# Autodesk Inventor assembly: ZB_Temperierstation
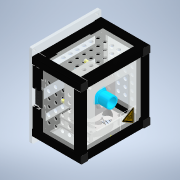
[picture p0: Inventor's stored thumbnail of the model, 180x180]
Saved by Autodesk Inventor 2022 (Build 260153000, 153)
## iProperties
Created: 2021-05-07
Part Number: ZB_Temperierstation
Document SubType Name: Assembly
Designer: Sebastian Seewald
Sending System: Autodesk Inventor 2021
Preprocessor: ST-DEVELOPER v18.1
Title: C:\Users\Sebastian Seewald\Documents\Inventor\Konstruktion_Studium\Projekt_1\Temperiereinheit\ZB\ZB_Temperierstation.stp
Author: Sebastian Seewald
## Documents named in this file (28)
- E:\Transfer\Sync\Hivemind\1-MCI-Unterlagen\Master\Semester 3\Projekt 2\011_Kartesischer_Roboter_Modul\07-CAD Files\03-Heizelement\ZB_Temperierstation.iam
- E:\Transfer\Sync\Hivemind\1-MCI-Unterlagen\Master\Semester 3\Projekt 2\011_Kartesischer_Roboter_Modul\07-CAD Files\03-Heizelement\0001_flasche.ipt
- E:\Transfer\Sync\Hivemind\1-MCI-Unterlagen\Master\Semester 3\Projekt 2\011_Kartesischer_Roboter_Modul\07-CAD Files\03-Heizelement\Temperierblock.ipt
- E:\Transfer\Sync\Hivemind\1-MCI-Unterlagen\Master\Semester 3\Projekt 2\011_Kartesischer_Roboter_Modul\07-CAD Files\03-Heizelement\Keramikhülse.ipt
- E:\Transfer\Sync\Hivemind\1-MCI-Unterlagen\Master\Semester 3\Projekt 2\011_Kartesischer_Roboter_Modul\07-CAD Files\03-Heizelement\ITEM_20x20_N2_200mm.ipt
- E:\Transfer\Sync\Hivemind\1-MCI-Unterlagen\Master\Semester 3\Projekt 2\011_Kartesischer_Roboter_Modul\07-CAD Files\03-Heizelement\Schutzglas.ipt
- E:\Transfer\Sync\Hivemind\1-MCI-Unterlagen\Master\Semester 3\Projekt 2\011_Kartesischer_Roboter_Modul\07-CAD Files\03-Heizelement\Schutzglas_oben.ipt
- E:\Transfer\Sync\Hivemind\1-MCI-Unterlagen\Master\Semester 3\Projekt 2\011_Kartesischer_Roboter_Modul\07-CAD Files\03-Heizelement\Schutzglas_Lüfter.ipt
- E:\Transfer\Sync\Hivemind\1-MCI-Unterlagen\Master\Semester 3\Projekt 2\011_Kartesischer_Roboter_Modul\07-CAD Files\03-Heizelement\3412ngh-rs0.ipt
- E:\Transfer\Sync\Hivemind\1-MCI-Unterlagen\Master\Semester 3\Projekt 2\011_Kartesischer_Roboter_Modul\07-CAD Files\03-Heizelement\Bimetallschalter.ipt
- E:\Transfer\Sync\Hivemind\1-MCI-Unterlagen\Master\Semester 3\Projekt 2\011_Kartesischer_Roboter_Modul\07-CAD Files\03-Heizelement\Distanzhülse.ipt
- E:\Transfer\Sync\Hivemind\1-MCI-Unterlagen\Master\Semester 3\Projekt 2\011_Kartesischer_Roboter_Modul\07-CAD Files\03-Heizelement\din_912-m4x0_7-35-10_9.ipt
- E:\Transfer\Sync\Hivemind\1-MCI-Unterlagen\Master\Semester 3\Projekt 2\011_Kartesischer_Roboter_Modul\07-CAD Files\03-Heizelement\mutter_din_934-m4x0_7.ipt
- E:\Transfer\Sync\Hivemind\1-MCI-Unterlagen\Master\Semester 3\Projekt 2\011_Kartesischer_Roboter_Modul\07-CAD Files\03-Heizelement\Schutzgitter.ipt
- E:\Transfer\Sync\Hivemind\1-MCI-Unterlagen\Master\Semester 3\Projekt 2\011_Kartesischer_Roboter_Modul\07-CAD Files\03-Heizelement\din_912-m3x0_5-6-10_9.ipt
- E:\Transfer\Sync\Hivemind\1-MCI-Unterlagen\Master\Semester 3\Projekt 2\011_Kartesischer_Roboter_Modul\07-CAD Files\03-Heizelement\HP_8x60_160W.ipt
- E:\Transfer\Sync\Hivemind\1-MCI-Unterlagen\Master\Semester 3\Projekt 2\011_Kartesischer_Roboter_Modul\07-CAD Files\03-Heizelement\Thermoelement.ipt
- E:\Transfer\Sync\Hivemind\1-MCI-Unterlagen\Master\Semester 3\Projekt 2\011_Kartesischer_Roboter_Modul\07-CAD Files\03-Heizelement\Abdeckkappe 5 20x20.ipt
- E:\Transfer\Sync\Hivemind\1-MCI-Unterlagen\Master\Semester 3\Projekt 2\011_Kartesischer_Roboter_Modul\07-CAD Files\03-Heizelement\Unterlegscheiben_Keramik.ipt
- E:\Transfer\Sync\Hivemind\1-MCI-Unterlagen\Master\Semester 3\Projekt 2\011_Kartesischer_Roboter_Modul\07-CAD Files\03-Heizelement\din_913-m4x10-c3.ipt
- E:\Transfer\Sync\Hivemind\1-MCI-Unterlagen\Master\Semester 3\Projekt 2\011_Kartesischer_Roboter_Modul\07-CAD Files\03-Heizelement\din_913-m4x8-a4.ipt
- E:\Transfer\Sync\Hivemind\1-MCI-Unterlagen\Master\Semester 3\Projekt 2\011_Kartesischer_Roboter_Modul\07-CAD Files\03-Heizelement\ITEM_20x20_N2_180mm.ipt
- E:\Transfer\Sync\Hivemind\1-MCI-Unterlagen\Master\Semester 3\Projekt 2\011_Kartesischer_Roboter_Modul\07-CAD Files\03-Heizelement\ITEM_20x20_N1_200mm.ipt
- E:\Transfer\Sync\Hivemind\1-MCI-Unterlagen\Master\Semester 3\Projekt 2\011_Kartesischer_Roboter_Modul\07-CAD Files\03-Heizelement\ITEM_20x20_200mm_Montage.ipt
- E:\Transfer\Sync\Hivemind\1-MCI-Unterlagen\Master\Semester 3\Projekt 2\011_Kartesischer_Roboter_Modul\07-CAD Files\03-Heizelement\Beilagscheibe_M5x1.ipt
- E:\Transfer\Sync\Hivemind\1-MCI-Unterlagen\Master\Semester 3\Projekt 2\011_Kartesischer_Roboter_Modul\07-CAD Files\03-Heizelement\ITEM_20x20_77mm.ipt
- E:\Transfer\Sync\Hivemind\1-MCI-Unterlagen\Master\Semester 3\Projekt 2\011_Kartesischer_Roboter_Modul\07-CAD Files\03-Heizelement\Kabeldurchführung.ipt
- E:\Transfer\Sync\Hivemind\1-MCI-Unterlagen\Master\Semester 3\Projekt 2\011_Kartesischer_Roboter_Modul\07-CAD Files\03-Heizelement\Heizelement_Grundplatte.ipt
## Components (73 placed, 27 different names)
1. Temperierblock:1 — Passend:48, Passend:176, Passend:177, Passend:178, Passend:179, Passend:180, Passend:181, Fluchtend:52, Fluchtend:53, Fluchtend:54, Fluchtend:55, Fluchtend:56, Fluchtend:57, Passend:182, Passend:184, Passend:187, Passend:188, Passend:189, Passend:231, Passend:251, Passend:258, Passend:259, Passend:260, Passend:261, Passend:262, Passend:263, Passend:264, Passend:303, Passend:304, Passend:305, Passend:306, Passend:307
2. Keramikhülse:1 — Passend:48, Passend:258, Passend:269, Passend:284
3. Keramikhülse:2 — Passend:263, Passend:264, Passend:265
4. Keramikhülse:3 — Passend:259, Passend:260, Passend:296
5. Keramikhülse:4 — Passend:261, Passend:262, Passend:266, Passend:288
6. Schutzglas:1 — Passend:212, Mate:249, Passend:250, Passend:308, Passend:309
7. Schutzglas:2 — Passend:215, Passend:245, Passend:246
8. Schutzglas:3 — Passend:214, Passend:247, Passend:248
9. ITEM_20x20_N2_200mm:8 — Passend:61, Passend:195, Passend:196, Fluchtend:63, Passend:240, Passend:241, Fluchtend:97, Passend:248
10. ITEM_20x20_N2_200mm:9 — Passend:62, Passend:193, Fluchtend:58, Fluchtend:60, Passend:242, Passend:243
11. ITEM_20x20_N2_200mm:10 — Passend:60, Passend:205, Fluchtend:76, Fluchtend:77, Passend:244
12. ITEM_20x20_N2_200mm:11 — Fluchtend:24, Passend:206, Fluchtend:78, Fluchtend:79, Passend:237, Passend:238, Passend:250
13. Schutzglas_oben:1 — Passend:60, Passend:61, Passend:62
14. Schutzglas_Lüfter:1 — Passend:118, Passend:119, Passend:120, Passend:121, Passend:122, Passend:123, Passend:124, Passend:129, Passend:130, Passend:131, Passend:132, Tangential:1, Passend:210, Passend:280, Passend:281
15. 3412ngh-rs0:1 — Passend:118, Passend:119, Passend:120, Passend:125, Passend:126, Passend:127, Passend:128, Passend:139, Passend:140, Passend:141, Passend:163
16. Bimetallschalter:1 — Passend:104, Passend:105, Passend:106, Passend:107, Passend:305
17. Distanzhülse:1 — Passend:121, Passend:126
18. Distanzhülse:2 — Passend:122, Passend:125
19. Distanzhülse:3 — Passend:123, Passend:128
20. Distanzhülse:4 — Passend:124, Passend:127
21. din_912-m4x0_7-35-10_9:1 — Passend:129, Tangential:2, Passend:135
22. din_912-m4x0_7-35-10_9:2 — Passend:132, Passend:134, Tangential:4, Passend:138
23. din_912-m4x0_7-35-10_9:3 — Passend:130, Passend:133, Tangential:3, Passend:136
24. din_912-m4x0_7-35-10_9:4 — Passend:131, Tangential:5, Passend:137
25. din_934-m4x0_7:1 — Passend:138, Passend:139
26. din_934-m4x0_7:2 — Passend:135, Passend:140
27. din_934-m4x0_7:3 — Passend:136, Passend:141
28. din_934-m4x0_7:4 — Passend:137, Passend:163
29. Schutzgitter:1 — Passend:133, Passend:134, Tangential:1, Tangential:2, Tangential:3, Tangential:4, Tangential:5
30. din_912-m3x0_5-6-10_9:1 — Passend:104, Passend:107, Passend:306
31. din_912-m3x0_5-6-10_9:2 — Passend:105, Passend:106, Passend:307
32. HP_8x60_160W:1 — Passend:176, Fluchtend:54, Tangential:6
33. HP_8x60_160W:2 — Passend:178, Fluchtend:57, Tangential:9
34. HP_8x60_160W:3 — Passend:177, Fluchtend:52, Tangential:7
35. HP_8x60_160W:4 — Passend:179, Fluchtend:55, Tangential:12
36. Thermoelement:1 — Passend:181, Fluchtend:53, Tangential:11
37. Thermoelement:2 — Passend:180, Fluchtend:56, Tangential:10
38. Abdeckkappe 5 20x20:1 — Passend:194, Fluchtend:61, Fluchtend:62
39. Abdeckkappe 5 20x20:2 — Fluchtend:24, Passend:207, Fluchtend:83, Fluchtend:84
40. Abdeckkappe 5 20x20:3 — Passend:209, Fluchtend:87, Fluchtend:88
41. Abdeckkappe 5 20x20:4 — Passend:208, Fluchtend:85, Fluchtend:86
42. Unterlegscheiben_Keramik:1 — Passend:275, Passend:294, Passend:297, Passend:302
43. Unterlegscheiben_Keramik:2 — Passend:274, Passend:295, Passend:299, Passend:300
44. Unterlegscheiben_Keramik:3 — Passend:273, Passend:289, Passend:290, Passend:298, Passend:301
45. Unterlegscheiben_Keramik:4 — Passend:272, Passend:291, Passend:292, Passend:293
46. din_913-m4x10-c3:2 — Passend:187, Tangential:9
47. din_913-m4x10-c3:4 — Passend:184, Tangential:7
48. din_913-m4x10-c3:5 — Passend:182, Tangential:6
49. din_913-m4x10-c3:6 — Passend:231, Tangential:12
50. din_913-m4x8-a4:1 — Passend:189, Tangential:11
51. din_913-m4x8-a4:2 — Passend:188, Tangential:10
52. ITEM_20x20_N2_180mm:1 — Passend:209, Fluchtend:87, Fluchtend:88, Passend:242, Passend:243, Passend:244, Passend:245, Passend:279, Fluchtend:101, Fluchtend:102, Mate:312
53. ITEM_20x20_N2_180mm:2 — Passend:193, Fluchtend:58, Fluchtend:60, Passend:194, Fluchtend:61, Fluchtend:62, Passend:195, Passend:196, Fluchtend:63, Passend:215, Passend:232, Fluchtend:89, Fluchtend:90, Passend:233, Fluchtend:91, Fluchtend:92, Mate:313
54. ITEM_20x20_N2_180mm:3 — Passend:207, Fluchtend:83, Fluchtend:84, Passend:214, Passend:237, Passend:238, Passend:240, Passend:241, Fluchtend:97, Passend:283, Fluchtend:105, Fluchtend:106
55. ITEM_20x20_N2_180mm:4 — Passend:205, Fluchtend:76, Fluchtend:77, Passend:206, Fluchtend:78, Fluchtend:79, Passend:208, Fluchtend:85, Fluchtend:86, Passend:210, Passend:212, Mate:249, Passend:280, Passend:282, Fluchtend:103, Fluchtend:104
56. ITEM_20x20_N1_200mm:1 — Passend:232, Fluchtend:89, Fluchtend:90, Passend:246, Passend:285, Passend:286, Fluchtend:107, Fluchtend:108, Mate:311
57. ITEM_20x20_N1_200mm:2 — Passend:279, Fluchtend:101, Fluchtend:102, Passend:281
58. ITEM_20x20_N1_200mm:3 — Passend:233, Fluchtend:91, Fluchtend:92, Passend:247, Passend:251, Mate:253
59. ITEM_20x20_200mm_Montage:1 — Mate:253, Passend:256, Passend:268, Passend:272, Passend:275, Passend:285, Fluchtend:108, Passend:291, Passend:292, Passend:294
60. ITEM_20x20_200mm_Montage:2 — Passend:257, Passend:267, Passend:273, Passend:274, Passend:286, Fluchtend:107, Passend:288, Passend:289, Passend:290, Passend:295
61. Beilagscheibe_M5x1:1 — Passend:256, Passend:269
62. Beilagscheibe_M5x1:2 — Passend:257, Passend:296
63. Beilagscheibe_M5x1:3 — Passend:265, Passend:268
64. Beilagscheibe_M5x1:4 — Passend:266, Passend:267
65. ITEM_20x20_77mm:1 — Passend:283, Fluchtend:105, Fluchtend:106
66. ITEM_20x20_77mm:2 — Passend:282, Fluchtend:103, Fluchtend:104, Passend:310
67. din_912-m4x0_7-35-10_9:5 — Passend:284, Passend:293
68. din_912-m4x0_7-35-10_9:6 — Passend:298, Passend:301
69. din_912-m4x0_7-35-10_9:7 — Passend:299, Passend:300
70. din_912-m4x0_7-35-10_9:8 — Passend:297, Passend:302
71. 0001_flasche:1 — Passend:303, Passend:304
72. Kabeldurchführung:1 — Passend:308, Passend:309, Passend:310
73. Heizelement_Grundplatte:1 — Mate:311, Mate:312, Mate:313
## Relationships (173: Mate 127, Flush 35, Tangent 11)
- Passend:48 [Mate]: Temperierblock:1 ↔ Keramikhülse:1
- Fluchtend:24 [Flush]: ITEM_20x20_N2_200mm:11 ↔ Abdeckkappe 5 20x20:2
- Passend:60 [Mate]: ITEM_20x20_N2_200mm:10 ↔ Schutzglas_oben:1
- Passend:61 [Mate]: ITEM_20x20_N2_200mm:8 ↔ Schutzglas_oben:1
- Passend:62 [Mate]: ITEM_20x20_N2_200mm:9 ↔ Schutzglas_oben:1
- Passend:104 [Mate]: Bimetallschalter:1 ↔ din_912-m3x0_5-6-10_9:1
- Passend:105 [Mate]: Bimetallschalter:1 ↔ din_912-m3x0_5-6-10_9:2
- Passend:106 [Mate]: Bimetallschalter:1 ↔ din_912-m3x0_5-6-10_9:2
- Passend:107 [Mate]: Bimetallschalter:1 ↔ din_912-m3x0_5-6-10_9:1
- Passend:118 [Mate]: Schutzglas_Lüfter:1 ↔ 3412ngh-rs0:1
- Passend:119 [Mate]: Schutzglas_Lüfter:1 ↔ 3412ngh-rs0:1
- Passend:120 [Mate]: Schutzglas_Lüfter:1 ↔ 3412ngh-rs0:1
- Passend:121 [Mate]: Schutzglas_Lüfter:1 ↔ Distanzhülse:1
- Passend:122 [Mate]: Schutzglas_Lüfter:1 ↔ Distanzhülse:2
- Passend:123 [Mate]: Schutzglas_Lüfter:1 ↔ Distanzhülse:3
- Passend:124 [Mate]: Schutzglas_Lüfter:1 ↔ Distanzhülse:4
- Passend:125 [Mate]: 3412ngh-rs0:1 ↔ Distanzhülse:2
- Passend:126 [Mate]: 3412ngh-rs0:1 ↔ Distanzhülse:1
- Passend:127 [Mate]: 3412ngh-rs0:1 ↔ Distanzhülse:4
- Passend:128 [Mate]: 3412ngh-rs0:1 ↔ Distanzhülse:3
- Passend:129 [Mate]: Schutzglas_Lüfter:1 ↔ din_912-m4x0_7-35-10_9:1
- Passend:130 [Mate]: Schutzglas_Lüfter:1 ↔ din_912-m4x0_7-35-10_9:3
- Passend:131 [Mate]: Schutzglas_Lüfter:1 ↔ din_912-m4x0_7-35-10_9:4
- Passend:132 [Mate]: Schutzglas_Lüfter:1 ↔ din_912-m4x0_7-35-10_9:2
- Passend:133 [Mate]: din_912-m4x0_7-35-10_9:3 ↔ Schutzgitter:1
- Passend:134 [Mate]: din_912-m4x0_7-35-10_9:2 ↔ Schutzgitter:1
- Tangential:1: Schutzglas_Lüfter:1 ↔ Schutzgitter:1
- Tangential:2: din_912-m4x0_7-35-10_9:1 ↔ Schutzgitter:1
- Tangential:3: din_912-m4x0_7-35-10_9:3 ↔ Schutzgitter:1
- Tangential:4: din_912-m4x0_7-35-10_9:2 ↔ Schutzgitter:1
- Tangential:5: din_912-m4x0_7-35-10_9:4 ↔ Schutzgitter:1
- Passend:135 [Mate]: din_912-m4x0_7-35-10_9:1 ↔ din_934-m4x0_7:2
- Passend:136 [Mate]: din_912-m4x0_7-35-10_9:3 ↔ din_934-m4x0_7:3
- Passend:137 [Mate]: din_912-m4x0_7-35-10_9:4 ↔ din_934-m4x0_7:4
- Passend:138 [Mate]: din_912-m4x0_7-35-10_9:2 ↔ din_934-m4x0_7:1
- Passend:139 [Mate]: 3412ngh-rs0:1 ↔ din_934-m4x0_7:1
- Passend:140 [Mate]: 3412ngh-rs0:1 ↔ din_934-m4x0_7:2
- Passend:141 [Mate]: 3412ngh-rs0:1 ↔ din_934-m4x0_7:3
- Passend:163 [Mate]: 3412ngh-rs0:1 ↔ din_934-m4x0_7:4
- Passend:176 [Mate]: Temperierblock:1 ↔ HP_8x60_160W:1
- Passend:177 [Mate]: Temperierblock:1 ↔ HP_8x60_160W:3
- Passend:178 [Mate]: Temperierblock:1 ↔ HP_8x60_160W:2
- Passend:179 [Mate]: Temperierblock:1 ↔ HP_8x60_160W:4
- Passend:180 [Mate]: Temperierblock:1 ↔ Thermoelement:2
- Passend:181 [Mate]: Temperierblock:1 ↔ Thermoelement:1
- Fluchtend:52 [Flush]: Temperierblock:1 ↔ HP_8x60_160W:3
- Fluchtend:53 [Flush]: Temperierblock:1 ↔ Thermoelement:1
- Fluchtend:54 [Flush]: Temperierblock:1 ↔ HP_8x60_160W:1
- Fluchtend:55 [Flush]: Temperierblock:1 ↔ HP_8x60_160W:4
- Fluchtend:56 [Flush]: Temperierblock:1 ↔ Thermoelement:2
- Fluchtend:57 [Flush]: Temperierblock:1 ↔ HP_8x60_160W:2
- Passend:182 [Mate]: Temperierblock:1 ↔ din_913-m4x10-c3:5
- Passend:184 [Mate]: Temperierblock:1 ↔ din_913-m4x10-c3:4
- Passend:187 [Mate]: Temperierblock:1 ↔ din_913-m4x10-c3:2
- Tangential:6: HP_8x60_160W:1 ↔ din_913-m4x10-c3:5
- Tangential:7: HP_8x60_160W:3 ↔ din_913-m4x10-c3:4
- Tangential:9: HP_8x60_160W:2 ↔ din_913-m4x10-c3:2
- Passend:188 [Mate]: Temperierblock:1 ↔ din_913-m4x8-a4:2
- Passend:189 [Mate]: Temperierblock:1 ↔ din_913-m4x8-a4:1
- Tangential:10: Thermoelement:2 ↔ din_913-m4x8-a4:2
- Tangential:11: Thermoelement:1 ↔ din_913-m4x8-a4:1
- Passend:193 [Mate]: ITEM_20x20_N2_200mm:9 ↔ ITEM_20x20_N2_180mm:2
- Fluchtend:58 [Flush]: ITEM_20x20_N2_200mm:9 ↔ ITEM_20x20_N2_180mm:2
- Fluchtend:60 [Flush]: ITEM_20x20_N2_200mm:9 ↔ ITEM_20x20_N2_180mm:2
- Passend:194 [Mate]: Abdeckkappe 5 20x20:1 ↔ ITEM_20x20_N2_180mm:2
- Fluchtend:61 [Flush]: Abdeckkappe 5 20x20:1 ↔ ITEM_20x20_N2_180mm:2
- Fluchtend:62 [Flush]: Abdeckkappe 5 20x20:1 ↔ ITEM_20x20_N2_180mm:2
- Passend:195 [Mate]: ITEM_20x20_N2_200mm:8 ↔ ITEM_20x20_N2_180mm:2
- Passend:196 [Mate]: ITEM_20x20_N2_200mm:8 ↔ ITEM_20x20_N2_180mm:2
- Fluchtend:63 [Flush]: ITEM_20x20_N2_200mm:8 ↔ ITEM_20x20_N2_180mm:2
- Passend:205 [Mate]: ITEM_20x20_N2_200mm:10 ↔ ITEM_20x20_N2_180mm:4
- Fluchtend:76 [Flush]: ITEM_20x20_N2_200mm:10 ↔ ITEM_20x20_N2_180mm:4
- Fluchtend:77 [Flush]: ITEM_20x20_N2_200mm:10 ↔ ITEM_20x20_N2_180mm:4
- Passend:206 [Mate]: ITEM_20x20_N2_200mm:11 ↔ ITEM_20x20_N2_180mm:4
- Fluchtend:78 [Flush]: ITEM_20x20_N2_200mm:11 ↔ ITEM_20x20_N2_180mm:4
- Fluchtend:79 [Flush]: ITEM_20x20_N2_200mm:11 ↔ ITEM_20x20_N2_180mm:4
- Passend:207 [Mate]: Abdeckkappe 5 20x20:2 ↔ ITEM_20x20_N2_180mm:3
- Fluchtend:83 [Flush]: Abdeckkappe 5 20x20:2 ↔ ITEM_20x20_N2_180mm:3
- Fluchtend:84 [Flush]: Abdeckkappe 5 20x20:2 ↔ ITEM_20x20_N2_180mm:3
- Passend:208 [Mate]: Abdeckkappe 5 20x20:4 ↔ ITEM_20x20_N2_180mm:4
- Fluchtend:85 [Flush]: Abdeckkappe 5 20x20:4 ↔ ITEM_20x20_N2_180mm:4
- Fluchtend:86 [Flush]: Abdeckkappe 5 20x20:4 ↔ ITEM_20x20_N2_180mm:4
- Passend:209 [Mate]: Abdeckkappe 5 20x20:3 ↔ ITEM_20x20_N2_180mm:1
- Fluchtend:87 [Flush]: Abdeckkappe 5 20x20:3 ↔ ITEM_20x20_N2_180mm:1
- Fluchtend:88 [Flush]: Abdeckkappe 5 20x20:3 ↔ ITEM_20x20_N2_180mm:1
- Passend:210 [Mate]: Schutzglas_Lüfter:1 ↔ ITEM_20x20_N2_180mm:4
- Passend:212 [Mate]: Schutzglas:1 ↔ ITEM_20x20_N2_180mm:4
- Passend:214 [Mate]: Schutzglas:3 ↔ ITEM_20x20_N2_180mm:3
- Passend:215 [Mate]: Schutzglas:2 ↔ ITEM_20x20_N2_180mm:2
- Passend:231 [Mate]: Temperierblock:1 ↔ din_913-m4x10-c3:6
- Tangential:12: HP_8x60_160W:4 ↔ din_913-m4x10-c3:6
- Passend:232 [Mate]: ITEM_20x20_N2_180mm:2 ↔ ITEM_20x20_N1_200mm:1
- Fluchtend:89 [Flush]: ITEM_20x20_N2_180mm:2 ↔ ITEM_20x20_N1_200mm:1
- Fluchtend:90 [Flush]: ITEM_20x20_N2_180mm:2 ↔ ITEM_20x20_N1_200mm:1
- Passend:233 [Mate]: ITEM_20x20_N2_180mm:2 ↔ ITEM_20x20_N1_200mm:3
- Fluchtend:91 [Flush]: ITEM_20x20_N2_180mm:2 ↔ ITEM_20x20_N1_200mm:3
- Fluchtend:92 [Flush]: ITEM_20x20_N2_180mm:2 ↔ ITEM_20x20_N1_200mm:3
- Passend:237 [Mate]: ITEM_20x20_N2_200mm:11 ↔ ITEM_20x20_N2_180mm:3
- Passend:238 [Mate]: ITEM_20x20_N2_200mm:11 ↔ ITEM_20x20_N2_180mm:3
- Passend:240 [Mate]: ITEM_20x20_N2_200mm:8 ↔ ITEM_20x20_N2_180mm:3
- Passend:241 [Mate]: ITEM_20x20_N2_200mm:8 ↔ ITEM_20x20_N2_180mm:3
- Fluchtend:97 [Flush]: ITEM_20x20_N2_200mm:8 ↔ ITEM_20x20_N2_180mm:3
- Passend:242 [Mate]: ITEM_20x20_N2_200mm:9 ↔ ITEM_20x20_N2_180mm:1
- Passend:243 [Mate]: ITEM_20x20_N2_200mm:9 ↔ ITEM_20x20_N2_180mm:1
- Passend:244 [Mate]: ITEM_20x20_N2_200mm:10 ↔ ITEM_20x20_N2_180mm:1
- Passend:245 [Mate]: Schutzglas:2 ↔ ITEM_20x20_N2_180mm:1
- Passend:246 [Mate]: Schutzglas:2 ↔ ITEM_20x20_N1_200mm:1
- Passend:247 [Mate]: Schutzglas:3 ↔ ITEM_20x20_N1_200mm:3
- Passend:248 [Mate]: Schutzglas:3 ↔ ITEM_20x20_N2_200mm:8
- Mate:249: Schutzglas:1 ↔ ITEM_20x20_N2_180mm:4
- Passend:250 [Mate]: Schutzglas:1 ↔ ITEM_20x20_N2_200mm:11
- Passend:251 [Mate] (40 mm): Temperierblock:1 ↔ ITEM_20x20_N1_200mm:3
- Mate:253 (37 mm): ITEM_20x20_N1_200mm:3 ↔ ITEM_20x20_200mm_Montage:1
- Passend:256 [Mate]: ITEM_20x20_200mm_Montage:1 ↔ Beilagscheibe_M5x1:1
- Passend:257 [Mate]: ITEM_20x20_200mm_Montage:2 ↔ Beilagscheibe_M5x1:2
- Passend:258 [Mate]: Temperierblock:1 ↔ Keramikhülse:1
- Passend:259 [Mate]: Temperierblock:1 ↔ Keramikhülse:3
- Passend:260 [Mate]: Temperierblock:1 ↔ Keramikhülse:3
- Passend:261 [Mate]: Temperierblock:1 ↔ Keramikhülse:4
- Passend:262 [Mate]: Temperierblock:1 ↔ Keramikhülse:4
- Passend:263 [Mate]: Temperierblock:1 ↔ Keramikhülse:2
- Passend:264 [Mate]: Temperierblock:1 ↔ Keramikhülse:2
- Passend:265 [Mate]: Keramikhülse:2 ↔ Beilagscheibe_M5x1:3
- Passend:266 [Mate]: Keramikhülse:4 ↔ Beilagscheibe_M5x1:4
- Passend:267 [Mate]: ITEM_20x20_200mm_Montage:2 ↔ Beilagscheibe_M5x1:4
- Passend:268 [Mate]: ITEM_20x20_200mm_Montage:1 ↔ Beilagscheibe_M5x1:3
- Passend:269 [Mate]: Keramikhülse:1 ↔ Beilagscheibe_M5x1:1
- Passend:272 [Mate]: Unterlegscheiben_Keramik:4 ↔ ITEM_20x20_200mm_Montage:1
- Passend:273 [Mate]: Unterlegscheiben_Keramik:3 ↔ ITEM_20x20_200mm_Montage:2
- Passend:274 [Mate]: Unterlegscheiben_Keramik:2 ↔ ITEM_20x20_200mm_Montage:2
- Passend:275 [Mate]: Unterlegscheiben_Keramik:1 ↔ ITEM_20x20_200mm_Montage:1
- Passend:279 [Mate]: ITEM_20x20_N2_180mm:1 ↔ ITEM_20x20_N1_200mm:2
- Fluchtend:101 [Flush]: ITEM_20x20_N2_180mm:1 ↔ ITEM_20x20_N1_200mm:2
- Fluchtend:102 [Flush]: ITEM_20x20_N2_180mm:1 ↔ ITEM_20x20_N1_200mm:2
- Passend:280 [Mate]: Schutzglas_Lüfter:1 ↔ ITEM_20x20_N2_180mm:4
- Passend:281 [Mate]: Schutzglas_Lüfter:1 ↔ ITEM_20x20_N1_200mm:2
- Passend:282 [Mate]: ITEM_20x20_N2_180mm:4 ↔ ITEM_20x20_77mm:2
- Fluchtend:103 [Flush]: ITEM_20x20_N2_180mm:4 ↔ ITEM_20x20_77mm:2
- Fluchtend:104 [Flush]: ITEM_20x20_N2_180mm:4 ↔ ITEM_20x20_77mm:2
- Passend:283 [Mate]: ITEM_20x20_N2_180mm:3 ↔ ITEM_20x20_77mm:1
- Fluchtend:105 [Flush]: ITEM_20x20_N2_180mm:3 ↔ ITEM_20x20_77mm:1
- Fluchtend:106 [Flush]: ITEM_20x20_N2_180mm:3 ↔ ITEM_20x20_77mm:1
- Passend:284 [Mate]: Keramikhülse:1 ↔ din_912-m4x0_7-35-10_9:5
- Passend:285 [Mate]: ITEM_20x20_N1_200mm:1 ↔ ITEM_20x20_200mm_Montage:1
- Passend:286 [Mate]: ITEM_20x20_N1_200mm:1 ↔ ITEM_20x20_200mm_Montage:2
- Fluchtend:107 [Flush]: ITEM_20x20_N1_200mm:1 ↔ ITEM_20x20_200mm_Montage:2
- Passend:288 [Mate]: Keramikhülse:4 ↔ ITEM_20x20_200mm_Montage:2
- Fluchtend:108 [Flush]: ITEM_20x20_N1_200mm:1 ↔ ITEM_20x20_200mm_Montage:1
- Passend:289 [Mate]: Unterlegscheiben_Keramik:3 ↔ ITEM_20x20_200mm_Montage:2
- Passend:290 [Mate]: Unterlegscheiben_Keramik:3 ↔ ITEM_20x20_200mm_Montage:2
- Passend:291 [Mate]: Unterlegscheiben_Keramik:4 ↔ ITEM_20x20_200mm_Montage:1
- Passend:292 [Mate]: Unterlegscheiben_Keramik:4 ↔ ITEM_20x20_200mm_Montage:1
- Passend:293 [Mate]: Unterlegscheiben_Keramik:4 ↔ din_912-m4x0_7-35-10_9:5
- Passend:294 [Mate]: Unterlegscheiben_Keramik:1 ↔ ITEM_20x20_200mm_Montage:1
- Passend:295 [Mate]: Unterlegscheiben_Keramik:2 ↔ ITEM_20x20_200mm_Montage:2
- Passend:296 [Mate]: Keramikhülse:3 ↔ Beilagscheibe_M5x1:2
- Passend:297 [Mate]: Unterlegscheiben_Keramik:1 ↔ din_912-m4x0_7-35-10_9:8
- Passend:298 [Mate]: Unterlegscheiben_Keramik:3 ↔ din_912-m4x0_7-35-10_9:6
- Passend:299 [Mate]: Unterlegscheiben_Keramik:2 ↔ din_912-m4x0_7-35-10_9:7
- Passend:300 [Mate]: Unterlegscheiben_Keramik:2 ↔ din_912-m4x0_7-35-10_9:7
- Passend:301 [Mate]: Unterlegscheiben_Keramik:3 ↔ din_912-m4x0_7-35-10_9:6
- Passend:302 [Mate]: Unterlegscheiben_Keramik:1 ↔ din_912-m4x0_7-35-10_9:8
- Passend:303 [Mate]: Temperierblock:1 ↔ 0001_flasche:1
- Passend:304 [Mate]: Temperierblock:1 ↔ 0001_flasche:1
- Passend:305 [Mate]: Temperierblock:1 ↔ Bimetallschalter:1
- Passend:306 [Mate]: Temperierblock:1 ↔ din_912-m3x0_5-6-10_9:1
- Passend:307 [Mate]: Temperierblock:1 ↔ din_912-m3x0_5-6-10_9:2
- Passend:308 [Mate]: Schutzglas:1 ↔ Kabeldurchführung:1
- Passend:309 [Mate]: Schutzglas:1 ↔ Kabeldurchführung:1
- Passend:310 [Mate]: ITEM_20x20_77mm:2 ↔ Kabeldurchführung:1
- Mate:311: ITEM_20x20_N1_200mm:1 ↔ Heizelement_Grundplatte:1
- Mate:312: ITEM_20x20_N2_180mm:1 ↔ Heizelement_Grundplatte:1
- Mate:313: ITEM_20x20_N2_180mm:2 ↔ Heizelement_Grundplatte:1
